# Autodesk Inventor assembly: pistonMechanism
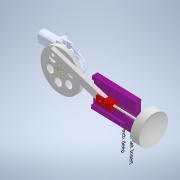
[picture p0: Inventor's stored thumbnail of the model, 180x180]
Saved by Autodesk Inventor 2020.2 (Build 242310000, 310)
## iProperties
Created: 2020-01-13
Part Number: pistonMechanism
Document SubType Name: Assembly
Designer: robst
Author: robst
## Documents named in this file (10)
- C:\git\CAD-Development\robSteele\2020BallTriggerMechanism\pistonMechanism.iam
- C:\git\CAD-Development\robSteele\2020BallTriggerMechanism\driveForPiston.ipt
- C:\git\CAD-Development\robSteele\2020BallTriggerMechanism\am-2235a Snow Blower Motor With Hex Shaft.iam
- C:\git\CAD-Development\robSteele\2020BallTriggerMechanism\am-2373 Snow Blower Motor Mount.ipt
- C:\git\CAD-Development\robSteele\2020BallTriggerMechanism\pistonHousing.ipt
- C:\git\CAD-Development\robSteele\2020BallTriggerMechanism\connectingRod.ipt
- C:\git\CAD-Development\robSteele\2020BallTriggerMechanism\piston.ipt
- C:\git\CAD-Development\robSteele\2020BallTriggerMechanism\93365A162_HEAT-SET INSERTS FOR PLASTICS.ipt
- C:\git\CAD-Development\robSteele\2020BallTriggerMechanism\plateForBall.ipt
- C:\git\CAD-Development\robSteele\2020BallTriggerMechanism\plateRod.ipt
## Components (11 placed, 9 different names)
1. driveForPiston:1 — Insert:3, Insert:4
2. am-2235a Snow Blower Motor With Hex Shaft:1 [sub-assembly] — Insert:1, Insert:2, Insert:3, Mate:1, Mate:3
3. am-2373 Snow Blower Motor Mount:1 — Insert:1, Insert:2
4. pistonHousing:1 — Mate:1, Mate:2, Flush:2, Mate:3, Mate:4, Flush:3, Flush:4
5. connectingRod:1 — Insert:4, Flush:1, Insert:5, Flush:2
6. piston:1 — Flush:1, Insert:5, Mate:2, Insert:6
7. 93365A162_HEAT-SET INSERTS FOR PLASTICS:1 — Insert:6, Insert:8
8. pistonHousing:2 — Mate:4, Flush:3, Flush:4
9. plateForBall:1 — Insert:7, Insert:9
10. 93365A162_HEAT-SET INSERTS FOR PLASTICS:2 — Insert:7
11. plateRod:1 — Insert:8, Insert:9
## Relationships (17: Insert 9, Flush 4, Mate 4)
- Insert:1: am-2235a Snow Blower Motor With Hex Shaft:1 ↔ am-2373 Snow Blower Motor Mount:1
- Insert:2: am-2235a Snow Blower Motor With Hex Shaft:1 ↔ am-2373 Snow Blower Motor Mount:1
- Insert:3: driveForPiston:1 ↔ am-2235a Snow Blower Motor With Hex Shaft:1
- Insert:4: driveForPiston:1 ↔ connectingRod:1
- Flush:1: connectingRod:1 ↔ piston:1
- Insert:5: connectingRod:1 ↔ piston:1
- Mate:1: am-2235a Snow Blower Motor With Hex Shaft:1 ↔ pistonHousing:1
- Mate:2: pistonHousing:1 ↔ piston:1
- Flush:2: pistonHousing:1 ↔ connectingRod:1
- Mate:3 (114.3 mm): am-2235a Snow Blower Motor With Hex Shaft:1 ↔ pistonHousing:1
- Insert:6: piston:1 ↔ 93365A162_HEAT-SET INSERTS FOR PLASTICS:1
- Mate:4: pistonHousing:1 ↔ pistonHousing:2
- Flush:3: pistonHousing:1 ↔ pistonHousing:2
- Flush:4: pistonHousing:1 ↔ pistonHousing:2
- Insert:7: plateForBall:1 ↔ 93365A162_HEAT-SET INSERTS FOR PLASTICS:2
- Insert:8 (-12.7 mm): 93365A162_HEAT-SET INSERTS FOR PLASTICS:1 ↔ plateRod:1
- Insert:9 (-12.7 mm): plateForBall:1 ↔ plateRod:1
